# Autodesk Inventor assembly: PidgeonIMU
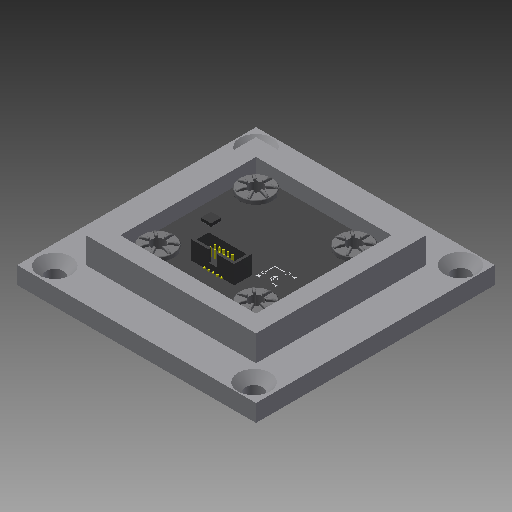
[picture p0: Inventor's stored thumbnail of the model, 512x512]
Saved by Autodesk Inventor 2019 (Build 230136000, 136)
## iProperties
Created: 2019-12-10
Part Number: PidgeonIMU
Document SubType Name: Assembly
Designer: james
Author: james
## Documents named in this file (3)
- F:\JimsRobot\FIRSTRobots\Design\Library\Jims\PidgeonIMU.iam
- F:\JimsRobot\FIRSTRobots\Design\Library\Jims\PigeonIMUMount.ipt
- F:\JimsRobot\FIRSTRobots\Design\Library\CTR\PIGEON_CAD\PIGEON_CAD\PIGEON.iam
## Components (2 placed, 2 different names)
1. PigeonIMUMount:1 — Mate:1, Mate:2
2. PIGEON:1 [sub-assembly] — Mate:1, Mate:2
## Relationships (2: Mate 2)
- Mate:1 (2.54 mm): PigeonIMUMount:1 ↔ PIGEON:1
- Mate:2: PigeonIMUMount:1 ↔ PIGEON:1
